# Autodesk Inventor assembly: Jar Jar
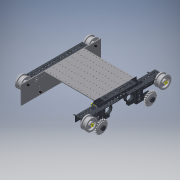
[picture p0: Inventor's stored thumbnail of the model, 180x180]
Saved by Autodesk Inventor 2016 (Build 200138000, 138)
## iProperties
Created: 2015-12-13
Part Number: Jar Jar
Document SubType Name: Assembly
Designer: tbloo
Author: tbloo
## Documents named in this file (18)
- C:\Users\TimB\Documents\GitHub\phi_robotics\3d-models\FTC_Tetrix_KOP_Block_Party\Tim Bloot Designs\JAr JaR Bot\BetaBot.iam
- C:\Users\TimB\Documents\GitHub\phi_robotics\3d-models\FTC_Tetrix_KOP_Block_Party\Tim Bloot Designs\Base Plate.ipt
- C:\Users\TimB\Documents\GitHub\phi_robotics\3d-models\FTC_Tetrix_KOP_Block_Party\Tetrix_Kit_FTC\Autodesk Inventor Files\tetrix_c_channel-3.ipt
- C:\Users\TimB\Documents\GitHub\phi_robotics\3d-models\FTC_Tetrix_KOP_Block_Party\Tetrix_Kit_FTC\Autodesk Inventor Files\tetrix_c_channel-2.ipt
- C:\Users\TimB\Documents\GitHub\phi_robotics\3d-models\FTC_Tetrix_KOP_Block_Party\Tetrix_Kit_FTC\Autodesk Inventor Files\tetrix_motor_mount-old.ipt
- C:\Users\TimB\Documents\GitHub\phi_robotics\3d-models\FTC_Tetrix_KOP_Block_Party\Tetrix_Kit_FTC\Autodesk Inventor Files\tetrix_bushing.ipt
- C:\Users\TimB\Documents\GitHub\phi_robotics\3d-models\FTC_Tetrix_KOP_Block_Party\Tim Bloot Designs\JAr JaR Bot\Tread Wheel Assembly.iam
- C:\Users\TimB\Documents\GitHub\phi_robotics\3d-models\FTC_Tetrix_KOP_Block_Party\Tetrix_Kit_FTC\Autodesk Inventor Files\tetrix_c_channel-round.ipt
- C:\Users\TimB\Documents\GitHub\phi_robotics\3d-models\FTC_Tetrix_KOP_Block_Party\Tetrix_Kit_FTC\Autodesk Inventor Files\tetrix_c_channel-1.ipt
- C:\Users\TimB\Documents\GitHub\phi_robotics\3d-models\FTC_Tetrix_KOP_Block_Party\Tim Bloot Designs\JAr JaR Bot\Tread Sproket Gear Assembly 2.iam
- C:\Users\TimB\Documents\GitHub\phi_robotics\3d-models\FTC_Tetrix_KOP_Block_Party\Tim Bloot Designs\JAr JaR Bot\tetrix_angle-144 MM.ipt
- C:\Users\TimB\Documents\GitHub\phi_robotics\3d-models\FTC_Tetrix_KOP_Block_Party\Tim Bloot Designs\JAr JaR Bot\inside Angle beam.ipt
- C:\Users\TimB\Documents\GitHub\phi_robotics\3d-models\FTC_Tetrix_KOP_Block_Party\Tetrix_Kit_FTC\Autodesk Inventor Files\tetrix_c_channel-4.ipt
- C:\Users\TimB\Documents\GitHub\phi_robotics\3d-models\FTC_Tetrix_KOP_Block_Party\Tetrix_Kit_FTC\Autodesk Inventor Files\tetrix_tread_wheel.ipt
- C:\Users\TimB\Documents\GitHub\phi_robotics\3d-models\FTC_Tetrix_KOP_Block_Party\Tim Bloot Designs\bot plate.ipt
- C:\Users\TimB\Documents\GitHub\phi_robotics\3d-models\FTC_Tetrix_KOP_Block_Party\Tetrix_Kit_FTC\Autodesk Inventor Files\tetrix_tread_sprocket_2012.ipt
- C:\Users\TimB\Documents\GitHub\phi_robotics\3d-models\FTC_Tetrix_KOP_Block_Party\Tetrix_Kit_FTC\Autodesk Inventor Files\tetrix_axle_lock.iam
- C:\Users\TimB\Documents\GitHub\phi_robotics\3d-models\FTC_Tetrix_KOP_Block_Party\Tetrix_Kit_FTC\Autodesk Inventor Files\tetrix_chain_gear-16t.ipt
## Components (49 placed, 17 different names)
1. Base Plate:1 — Rigid:117, Rigid:137, Mate:1, Flush:3
2. tetrix_motor_mount-old:6 — Rigid:147
3. tetrix_motor_mount-old:8 — Rigid:148
4. tetrix_c_channel-3:5 — Rigid:116, Rigid:133, Rigid:136, Rigid:139
5. tetrix_c_channel-2:19 — Rigid:115, Rigid:135
6. tetrix_c_channel-2:20 — Rigid:134
7. tetrix_c_channel-2:21 — Rigid:131
8. tetrix_motor_mount-old:9
9. Tread Wheel Assembly:7 [sub-assembly]
10. Tread Wheel Assembly:8 [sub-assembly]
11. tetrix_c_channel-round:4
12. tetrix_c_channel-1:4
13. tetrix_bushing:19
14. tetrix_bushing:20
15. tetrix_c_channel-2:22 — Rigid:132, Rigid:138
16. tetrix_motor_mount-old:10
17. tetrix_c_channel-round:5
18. tetrix_c_channel-1:5
19. tetrix_bushing:21
20. tetrix_bushing:22
21. Tread Sproket Gear Assembly 2:3 [sub-assembly]
22. Tread Sproket Gear Assembly 2:4 [sub-assembly]
23. inside Angle beam:1 — Rigid:137, Rigid:138, Rigid:139
24. inside Angle beam:2 — Rigid:115, Rigid:116, Rigid:117
25. tetrix_angle-144 MM:3 — Rigid:134, Rigid:135, Rigid:136
26. tetrix_angle-144 MM:4 — Rigid:131, Rigid:132, Rigid:133
27. tetrix_c_channel-4:1 — Rigid:140, Rigid:146
28. tetrix_tread_wheel:1 — Rotational:54, Rotational:55
29. bot plate:1 — Rigid:140, Rotational:56, Mate:1, Flush:3, Rotational:63, Rotational:65, Rotational:69
30. tetrix_bushing:23 — Rotational:54, Rotational:57
31. tetrix_bushing:24 — Rotational:55, Rotational:58
32. tetrix_bushing:25 — Rotational:56, Rotational:57
33. tetrix_bushing:26 — Rotational:58
34. tetrix_tread_wheel:3
35. tetrix_bushing:27
36. tetrix_bushing:28
37. tetrix_bushing:29
38. tetrix_bushing:30 — Rotational:63
39. tetrix_tread_sprocket_2012:1 — Rigid:150, Rigid:151
40. tetrix_chain_gear-16t:1 — Rigid:150, Rotational:64
41. tetrix_bushing:31 — Rotational:65, Rotational:66
42. tetrix_bushing:32 — Rotational:64
43. tetrix_c_channel-round:6 — Rigid:146, Rigid:147, Rigid:148
44. tetrix_axle_lock:2 [sub-assembly] — Rigid:151, Rotational:66
45. tetrix_tread_sprocket_2012:2
46. tetrix_chain_gear-16t:2
47. tetrix_bushing:33 — Rotational:69
48. tetrix_bushing:34
49. tetrix_axle_lock:3 [sub-assembly]
## Relationships (52: WeldJoint 26, RevoluteJoint 24, Mate 1, Flush 1)
- [WeldJoint]: tetrix_c_channel-2:19 ↔ tetrix_motor_mount-old:9
- [RevoluteJoint]: tetrix_c_channel-2:20 ↔ Tread Wheel Assembly:7
- [RevoluteJoint]: tetrix_c_channel-2:21 ↔ Tread Wheel Assembly:8
- [WeldJoint]: tetrix_c_channel-2:19 ↔ tetrix_c_channel-round:4
- [WeldJoint]: tetrix_c_channel-round:4 ↔ tetrix_c_channel-1:4
- [RevoluteJoint]: tetrix_c_channel-1:4 ↔ tetrix_bushing:19
- [RevoluteJoint]: tetrix_c_channel-1:4 ↔ tetrix_bushing:20
- [WeldJoint]: tetrix_c_channel-2:22 ↔ tetrix_motor_mount-old:10
- [WeldJoint]: tetrix_c_channel-2:22 ↔ tetrix_c_channel-round:5
- [WeldJoint]: tetrix_c_channel-round:5 ↔ tetrix_c_channel-1:5
- [RevoluteJoint]: tetrix_c_channel-1:5 ↔ tetrix_bushing:21
- [RevoluteJoint]: tetrix_c_channel-1:5 ↔ tetrix_bushing:22
- [RevoluteJoint]: tetrix_bushing:19 ↔ Tread Sproket Gear Assembly 2:3
- [RevoluteJoint]: tetrix_bushing:22 ↔ Tread Sproket Gear Assembly 2:4
- Rigid:115 [WeldJoint]: tetrix_c_channel-2:19 ↔ inside Angle beam:2
- Rigid:116 [WeldJoint]: tetrix_c_channel-3:5 ↔ inside Angle beam:2
- Rigid:117 [WeldJoint]: Base Plate:1 ↔ inside Angle beam:2
- Rigid:131 [WeldJoint]: tetrix_c_channel-2:21 ↔ tetrix_angle-144 MM:4
- Rigid:132 [WeldJoint]: tetrix_c_channel-2:22 ↔ tetrix_angle-144 MM:4
- Rigid:133 [WeldJoint]: tetrix_c_channel-3:5 ↔ tetrix_angle-144 MM:4
- Rigid:134 [WeldJoint]: tetrix_c_channel-2:20 ↔ tetrix_angle-144 MM:3
- Rigid:135 [WeldJoint]: tetrix_c_channel-2:19 ↔ tetrix_angle-144 MM:3
- Rigid:136 [WeldJoint]: tetrix_c_channel-3:5 ↔ tetrix_angle-144 MM:3
- Rigid:137 [WeldJoint]: Base Plate:1 ↔ inside Angle beam:1
- Rigid:138 [WeldJoint]: tetrix_c_channel-2:22 ↔ inside Angle beam:1
- Rigid:139 [WeldJoint]: tetrix_c_channel-3:5 ↔ inside Angle beam:1
- Rigid:140 [WeldJoint]: tetrix_c_channel-4:1 ↔ bot plate:1
- Rotational:54 [RevoluteJoint]: tetrix_tread_wheel:1 ↔ tetrix_bushing:23
- Rotational:55 [RevoluteJoint]: tetrix_tread_wheel:1 ↔ tetrix_bushing:24
- Rotational:56 [RevoluteJoint]: bot plate:1 ↔ tetrix_bushing:25
- Rotational:57 [RevoluteJoint]: tetrix_bushing:23 ↔ tetrix_bushing:25
- Rotational:58 [RevoluteJoint]: tetrix_bushing:24 ↔ tetrix_bushing:26
- Mate:1: Base Plate:1 ↔ bot plate:1
- Flush:3: Base Plate:1 ↔ bot plate:1
- [RevoluteJoint]: tetrix_tread_wheel:3 ↔ tetrix_bushing:27
- [RevoluteJoint]: tetrix_tread_wheel:3 ↔ tetrix_bushing:28
- [RevoluteJoint]: tetrix_bushing:27 ↔ tetrix_bushing:29
- [RevoluteJoint]: tetrix_bushing:28 ↔ tetrix_bushing:30
- Rotational:63 [RevoluteJoint]: bot plate:1 ↔ tetrix_bushing:30
- Rigid:146 [WeldJoint]: tetrix_c_channel-4:1 ↔ tetrix_c_channel-round:6
- Rigid:147 [WeldJoint]: tetrix_motor_mount-old:6 ↔ tetrix_c_channel-round:6
- Rigid:148 [WeldJoint]: tetrix_motor_mount-old:8 ↔ tetrix_c_channel-round:6
- Rigid:150 [WeldJoint]: tetrix_tread_sprocket_2012:1 ↔ tetrix_chain_gear-16t:1
- Rigid:151 [WeldJoint]: tetrix_tread_sprocket_2012:1 ↔ tetrix_axle_lock:2
- Rotational:64 [RevoluteJoint]: tetrix_chain_gear-16t:1 ↔ tetrix_bushing:32
- Rotational:65 [RevoluteJoint]: bot plate:1 ↔ tetrix_bushing:31
- Rotational:66 [RevoluteJoint]: tetrix_bushing:31 ↔ tetrix_axle_lock:2
- [WeldJoint]: tetrix_tread_sprocket_2012:2 ↔ tetrix_chain_gear-16t:2
- [WeldJoint]: tetrix_tread_sprocket_2012:2 ↔ tetrix_axle_lock:3
- [RevoluteJoint]: tetrix_chain_gear-16t:2 ↔ tetrix_bushing:34
- [RevoluteJoint]: tetrix_bushing:33 ↔ tetrix_axle_lock:3
- Rotational:69 [RevoluteJoint]: bot plate:1 ↔ tetrix_bushing:33
## Named parameters: d210_d112_d58_d39 = 0 mm, d211_d113_d59_d40 = -5.431137 deg, d212_d170 = 0 mm, d213_d171 = 0 deg, d221_d137 = 0 mm, d222_d138 = 0 mm, d223_d139 = 0 mm, d224_d140 = 0.202797 deg, d225_d141 = 0 mm, d226_d142 = 0 deg, d227_d153_d150_d116_d65_d11 = 0 mm, d228_d154_d143_d137 = 0 mm, d229_d155_d144_d138 = 0 mm, d230_d156_d145_d139 = 0 mm, d231_d157_d146_d140 = 0 deg, d232_d158_d147_d141 = 0 mm, d233_d159_d148_d142 = 0 deg, d238_d168 = 0 mm, d239_d169 = -0.202797 deg, d240_d114_d60_d41 = 0 mm, d241_d115_d61_d42 = 0.840635 deg, d242_d116_d65_d11 = 0 mm, d379_d367 = 0 mm, d380_d368 = 30.349775 deg, d381_d369 = 0 mm, d382_d370 = 0.976308 deg, d383_d373 = 0 mm, d384_d374 = -18.241546 deg, d385_d375 = 0 mm, d386_d376 = -1.667601 deg, d422_d412 = 0 mm, d423_d415 = 0 mm, d424_d416 = 0 mm, d425_d417 = 0 deg, d426_d420 = 0 mm, d427_d421 = 157.367765 deg
